# Autodesk Inventor assembly: Assembly1
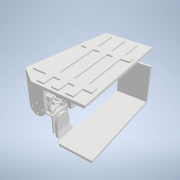
[picture p0: Inventor's stored thumbnail of the model, 180x180]
Saved by Autodesk Inventor 2020 (Build 240168000, 168)
## iProperties
Created: 2019-12-29
Part Number: Assembly1
Document SubType Name: Assembly
Designer: tdmp4
Author: tdmp4
## Documents named in this file (7)
- C:\Users\tdmp4\OneDrive\Documents\GitHub\CAD-2020\Assembly1.iam
- C:\Users\tdmp4\OneDrive\Documents\GitHub\CAD-2020\ServoCity\637112.ipt
- C:\Users\tdmp4\OneDrive\Documents\GitHub\CAD-2020\RevRobotics\REV-41-1097.ipt
- C:\Users\tdmp4\OneDrive\Documents\GitHub\CAD-2020\ServoCity\585422.ipt
- C:\Users\tdmp4\OneDrive\Documents\GitHub\CAD-2020\ServoCity\585424.ipt
- C:\Users\tdmp4\OneDrive\Documents\GitHub\CAD-2020\Intake\Part1.ipt
- C:\Users\tdmp4\OneDrive\Documents\GitHub\CAD-2020\Intake\gripperMove.ipt
## Components (7 placed, 6 different names)
1. 637112:1 — Mate:1, Mate:2, Mate:3, Mate:4, Mate:5, Mate:6
2. 637112:2 — Mate:7, Mate:8, Mate:9, Mate:10, Mate:11, Mate:12, Mate:16, Mate:17
3. REV-41-1097:1 — Mate:1, Mate:2, Mate:3
4. 585422:1 — Mate:4, Mate:5, Mate:6, Mate:7, Mate:8, Mate:9
5. 585424:1 — Mate:10, Mate:11, Mate:12, Mate:13, Mate:14, Mate:15
6. Part1:1 — Mate:13, Mate:14, Mate:15
7. gripperMove:1 — Mate:16, Mate:17
## Relationships (17: Mate 17)
- Mate:1: 637112:1 ↔ REV-41-1097:1
- Mate:2: 637112:1 ↔ REV-41-1097:1
- Mate:3: 637112:1 ↔ REV-41-1097:1
- Mate:4: 637112:1 ↔ 585422:1
- Mate:5: 637112:1 ↔ 585422:1
- Mate:6: 637112:1 ↔ 585422:1
- Mate:7: 637112:2 ↔ 585422:1
- Mate:8: 637112:2 ↔ 585422:1
- Mate:9: 637112:2 ↔ 585422:1
- Mate:10: 637112:2 ↔ 585424:1
- Mate:11: 637112:2 ↔ 585424:1
- Mate:12: 637112:2 ↔ 585424:1
- Mate:13: 585424:1 ↔ Part1:1
- Mate:14: 585424:1 ↔ Part1:1
- Mate:15: 585424:1 ↔ Part1:1
- Mate:16: 637112:2 ↔ gripperMove:1
- Mate:17: 637112:2 ↔ gripperMove:1
